# Autodesk Inventor assembly: camera_assembly
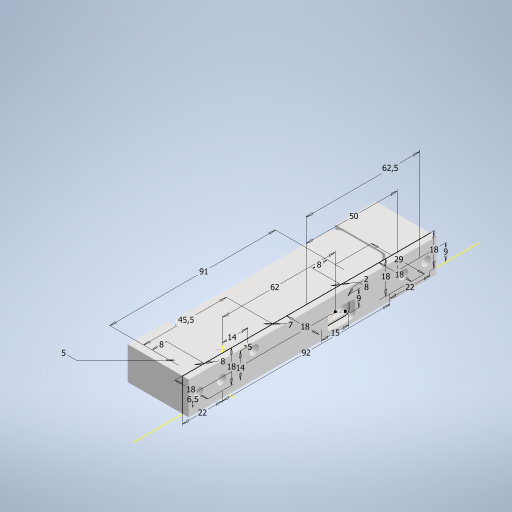
[picture p0: Inventor's stored thumbnail of the model, 512x512]
Saved by Autodesk Inventor 2024.3 (Build 283343000, 343)
## iProperties
Created: 2026-05-03
Part Number: camera_assembly
Document SubType Name: Assembly
Designer: owozn
Author: owozn
## Documents named in this file (3)
- C:\Users\owozn\Documents\Nauka\Studia\mgr\Semestr_3\Magisterka\uMule\mechanics\subsets\attachments\camera\camera_assembly.iam
- C:\Users\owozn\Documents\Nauka\Studia\mgr\Semestr_3\Magisterka\uMule\mechanics\subsets\attachments\camera\camera_holder.ipt
- C:\Users\owozn\Documents\Nauka\Studia\mgr\Semestr_3\Magisterka\uMule\mechanics\subsets\attachments\camera\camera_model.ipt
## Components (2 placed, 2 different names)
1. camera_holder:1 — Mate:1, Mate:2
2. camera_model:1 — Mate:1, Mate:2
## Relationships (2: Mate 2)
- Mate:1: camera_holder:1 ↔ camera_model:1
- Mate:2: camera_holder:1 ↔ camera_model:1
